# Autodesk Inventor assembly: Mounting_ID6_ASM
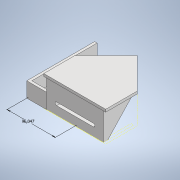
[picture p0: Inventor's stored thumbnail of the model, 180x180]
Saved by Autodesk Inventor 2022.2 (Build 262287010, 287A)
## iProperties
Created: 2024-09-30
Part Number: Mounting_ID6_ASM
Document SubType Name: Assembly
Designer: ppovolni
Author: ppovolni
## Documents named in this file (3)
- D:\3_Local_Projekte\ALF\alf_nmr_magnetometer\2_Project_Motiontracking_Robotarm\Marker\Mounting_ID6_ASM.iam
- D:\3_Local_Projekte\ALF\alf_nmr_magnetometer\2_Project_Motiontracking_Robotarm\Marker\Mounting_ID6.ipt
- D:\3_Local_Projekte\ALF\alf_nmr_magnetometer\2_Project_Motiontracking_Robotarm\Marker\Mounting_ID6_Support.ipt
## Components (2 placed, 2 different names)
1. Mounting_ID6:1 — Fluchtend:1, Fluchtend:2, Passend:1
2. Mounting_ID6_Support:1 — Fluchtend:1, Fluchtend:2, Passend:1
## Relationships (3: Flush 2, Mate 1)
- Fluchtend:1 [Flush]: Mounting_ID6:1 ↔ Mounting_ID6_Support:1
- Fluchtend:2 [Flush]: Mounting_ID6:1 ↔ Mounting_ID6_Support:1
- Passend:1 [Mate]: Mounting_ID6:1 ↔ Mounting_ID6_Support:1
